# Autodesk Inventor assembly: Robot
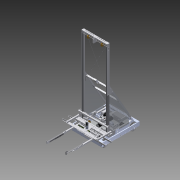
[picture p0: Inventor's stored thumbnail of the model, 180x180]
Saved by Autodesk Inventor 2015 (Build 190159000, 159)
## iProperties
Created: 2015-01-17
Part Number: Robot
Document SubType Name: Assembly
Designer: Jarod
Author: Jarod
## Documents named in this file (12)
- C:\Users\Jarod\Documents\Robotics\FRC\2015\CAD\Robot\Robot.iam
- C:\Users\Jarod\Documents\Robotics\FRC\2015\CAD\Robot\Chassis\Chassis.iam
- C:\Users\Jarod\Documents\Robotics\FRC\2015\CAD\Robot\Vertical Lift\Vertical Lift.iam
- C:\Users\Jarod\Documents\Robotics\FRC\2015\CAD\Robot\Lift Cart\Lift Cart.iam
- C:\Users\Jarod\Documents\Robotics\FRC\2015\CAD\Robot\Pickup Arms\Pickup Arm Left.iam
- C:\Users\Jarod\Documents\Robotics\FRC\2015\CAD\Robot\Pickup Arms\Pickup Arm Right.iam
- C:\Users\Jarod\Documents\Robotics\FRC\2015\CAD\Robot\tote.iam
- C:\Users\Jarod\Documents\Robotics\FRC\2015\CAD\Robot\bin.iam
- C:\Users\Jarod\Documents\Robotics\FRC\2015\CAD\Robot\Noodle Sucker\Noodle Sucker.iam
- C:\Users\Jarod\Documents\Robotics\FRC\2015\CAD\Robot\noodle.ipt
- C:\Users\Jarod\Documents\Robotics\FRC\2015\CAD\front slider guard.ipt
- C:\Users\Jarod\Documents\Robotics\FRC\2015\CAD\gusset guard.ipt
## Components (18 placed, 11 different names)
1. Chassis:1 [sub-assembly] — Mate:17, Mate:18, Mate:19
2. Vertical Lift:1 [sub-assembly] — Mate:6, Mate:7, Mate:8, Mate:17, Mate:18, Mate:19, Mate:22, Mate:29
3. Lift Cart:1 [sub-assembly] — Mate:6, Mate:7, Mate:8, Mate:11, Mate:14, Mate:15, Mate:16, Mate:20, Mate:21, Mate:39, Mate:40, Flush:3
4. Pickup Arm Left:1 [sub-assembly] — Mate:11, Mate:16, Mate:21, Mate:36, Mate:37, Mate:38
5. Pickup Arm Right:1 [sub-assembly] — Mate:14, Mate:15, Mate:20
6. Noodle Sucker:1 [sub-assembly] — Mate:22, Mate:29, Mate:24, Mate:25, Mate:26, Mate:27
7. tote:1 [sub-assembly]
8. tote:2 [sub-assembly] — Flush:1, Flush:2, Mate:28
9. tote:3 [sub-assembly] — Flush:1, Flush:2, Mate:28
10. bin:1 [sub-assembly]
11. bin:2 [sub-assembly]
12. bin:3 [sub-assembly]
13. noodle:1 — Mate:24
14. noodle:2 — Mate:25
15. noodle:3 — Mate:26
16. noodle:4 — Mate:27
17. front slider guard:1 — Mate:39, Mate:40, Flush:3
18. gusset guard:1 — Mate:36, Mate:37, Mate:38
## Relationships (27: Mate 24, Flush 3)
- Mate:6 (25.4 mm): Vertical Lift:1 ↔ Lift Cart:1
- Mate:7 (25.4 mm): Vertical Lift:1 ↔ Lift Cart:1
- Mate:8 (6.35 mm): Vertical Lift:1 ↔ Lift Cart:1
- Mate:11 (6.0452 mm): Lift Cart:1 ↔ Pickup Arm Left:1
- Mate:14 (6.0452 mm): Lift Cart:1 ↔ Pickup Arm Right:1
- Mate:15: Lift Cart:1 ↔ Pickup Arm Right:1
- Mate:16: Lift Cart:1 ↔ Pickup Arm Left:1
- Mate:17: Chassis:1 ↔ Vertical Lift:1
- Mate:18: Chassis:1 ↔ Vertical Lift:1
- Mate:19: Chassis:1 ↔ Vertical Lift:1
- Mate:20 (100.0125 mm): Lift Cart:1 ↔ Pickup Arm Right:1
- Mate:21 (100.0125 mm): Lift Cart:1 ↔ Pickup Arm Left:1
- Mate:22: Vertical Lift:1 ↔ Noodle Sucker:1
- Mate:29: Vertical Lift:1 ↔ Noodle Sucker:1
- Mate:24 (82.55 mm): Noodle Sucker:1 ↔ noodle:1
- Mate:25 (82.55 mm): Noodle Sucker:1 ↔ noodle:2
- Mate:26 (82.55 mm): Noodle Sucker:1 ↔ noodle:3
- Mate:27 (82.55 mm): Noodle Sucker:1 ↔ noodle:4
- Flush:1: tote:2 ↔ tote:3
- Flush:2: tote:2 ↔ tote:3
- Mate:28: tote:2 ↔ tote:3
- Mate:36: Pickup Arm Left:1 ↔ gusset guard:1
- Mate:37: Pickup Arm Left:1 ↔ gusset guard:1
- Mate:38: Pickup Arm Left:1 ↔ gusset guard:1
- Mate:39: Lift Cart:1 ↔ front slider guard:1
- Mate:40: Lift Cart:1 ↔ front slider guard:1
- Flush:3: Lift Cart:1 ↔ front slider guard:1
